# Autodesk Inventor assembly: PLANCHAS PARA CORTAR
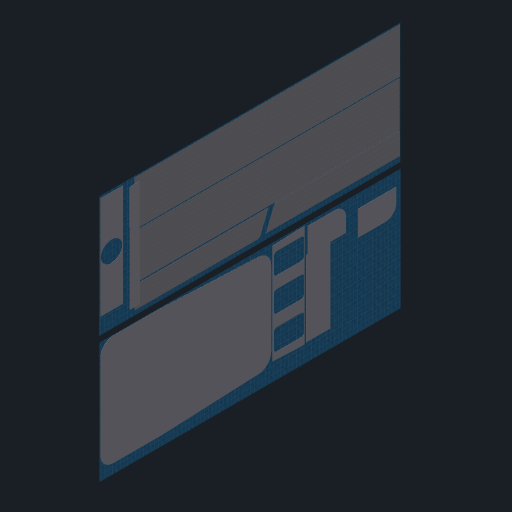
[picture p0: Inventor's stored thumbnail of the model, 512x512]
Saved by Autodesk Inventor 2024.3 (Build 283343000, 343)
## iProperties
Created: 2024-05-15
Part Number: PLANCHAS PARA CORTAR
Material: Generic
Document SubType Name: Assembly
Designer: Niler
Author: Niler
## Documents named in this file (10)
- C:\Users\Niler\OneDrive\Escritorio\RECICLADOR\RECICLADOR_MODELO_3D\PIEZAS\PLANCHAS PARA CORTAR.iam
- C:\Users\Niler\OneDrive\Escritorio\RECICLADOR\RECICLADOR_MODELO_3D\PIEZAS\PLANCHA_COMPLETA.ipt
- C:\Users\Niler\OneDrive\Escritorio\RECICLADOR\RECICLADOR_MODELO_3D\PIEZAS\CARCASA_ALUM_4.ipt
- C:\Users\Niler\OneDrive\Escritorio\RECICLADOR\RECICLADOR_MODELO_3D\PIEZAS\CARCASA_ALUM_2.ipt
- C:\Users\Niler\OneDrive\Escritorio\RECICLADOR\RECICLADOR_MODELO_3D\PIEZAS\CARCASA_ALUM_2_FLAT.ipt
- C:\Users\Niler\OneDrive\Escritorio\RECICLADOR\RECICLADOR_MODELO_3D\PIEZAS\CARCASA_ALUM_1_FLAT.ipt
- C:\Users\Niler\OneDrive\Escritorio\RECICLADOR\RECICLADOR_MODELO_3D\PIEZAS\CARCASA_ALUM_5.ipt
- C:\Users\Niler\OneDrive\Escritorio\RECICLADOR\RECICLADOR_MODELO_3D\PIEZAS\CARCASA_ALUM_6.ipt
- C:\Users\Niler\OneDrive\Escritorio\RECICLADOR\RECICLADOR_MODELO_3D\PIEZAS\CARCASA_ALUM_7.ipt
- C:\Users\Niler\OneDrive\Escritorio\RECICLADOR\RECICLADOR_MODELO_3D\PIEZAS\CARCASA_ALUM_8.ipt
## Components (13 placed, 9 different names)
1. PLANCHA_COMPLETA:1 — Mate:1, Mate:2, Mate:3
2. CARCASA_ALUM_4:1 — Mate:1
3. CARCASA_ALUM_2:1 — Mate:8
4. PLANCHA_COMPLETA:2 — Mate:4, Mate:5, Mate:6, Mate:7, Mate:8
5. CARCASA_ALUM_1_FLAT:1 — Mate:4
6. CARCASA_ALUM_1_FLAT:2 — Mate:5
7. CARCASA_ALUM_2_FLAT:4 — Mate:6
8. CARCASA_ALUM_2_FLAT:5 — Mate:7
9. CARCASA_ALUM_5:1 — Mate:2
10. CARCASA_ALUM_6:1
11. CARCASA_ALUM_6:2
12. CARCASA_ALUM_7:1 — Mate:3
13. CARCASA_ALUM_8:1
## Relationships (8: Mate 8)
- Mate:1: PLANCHA_COMPLETA:1 ↔ CARCASA_ALUM_4:1
- Mate:2: PLANCHA_COMPLETA:1 ↔ CARCASA_ALUM_5:1
- Mate:3: PLANCHA_COMPLETA:1 ↔ CARCASA_ALUM_7:1
- Mate:4: PLANCHA_COMPLETA:2 ↔ CARCASA_ALUM_1_FLAT:1
- Mate:5: PLANCHA_COMPLETA:2 ↔ CARCASA_ALUM_1_FLAT:2
- Mate:6: PLANCHA_COMPLETA:2 ↔ CARCASA_ALUM_2_FLAT:4
- Mate:7: PLANCHA_COMPLETA:2 ↔ CARCASA_ALUM_2_FLAT:5
- Mate:8: CARCASA_ALUM_2:1 ↔ PLANCHA_COMPLETA:2
